# Autodesk Inventor assembly: ASY MSC Жабры
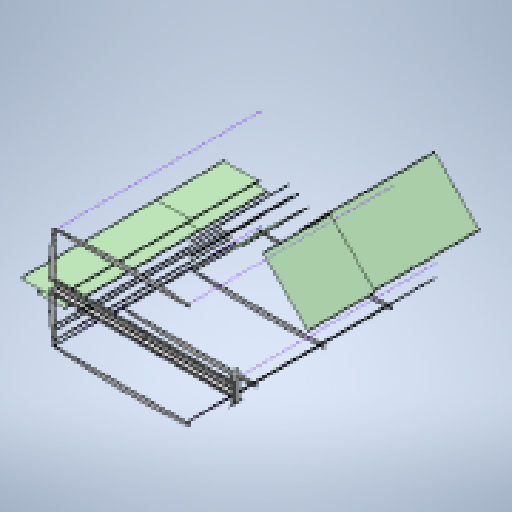
[picture p0: Inventor's stored thumbnail of the model, 512x512]
Saved by Autodesk Inventor 2025 (Build 290162010, 162A)
## iProperties
Created: 2024-08-31
Part Number: ASY MSC Жабры
Document SubType Name: Assembly
Designer: pokla
Author: pokla
## Documents named in this file (24)
- C:\Users\admin\YandexDisk-badmisterfox\домашниий пк\Inventor\Manturovo\Manturovo_Se-clar\ASY MSC Жабры.iam
- C:\Users\admin\YandexDisk-badmisterfox\домашниий пк\Inventor\Manturovo\Manturovo_Se-clar\MSC 0101 sheet gills.ipt
- C:\Users\admin\YandexDisk-badmisterfox\домашниий пк\Inventor\Manturovo\Manturovo_Se-clar\MSC 081 pillar 1.ipt
- C:\Users\admin\YandexDisk-badmisterfox\домашниий пк\Inventor\Manturovo\Manturovo_Se-clar\MSC 0102 sheet gills.ipt
- C:\Users\admin\YandexDisk-badmisterfox\домашниий пк\Inventor\Manturovo\Manturovo_Se-clar\MSC 0202 sheet gills.ipt
- C:\Users\admin\YandexDisk-badmisterfox\домашниий пк\Inventor\Manturovo\Manturovo_Se-clar\MSC 0103 sheet gills.ipt
- C:\Users\admin\YandexDisk-badmisterfox\домашниий пк\Inventor\Manturovo\Manturovo_Se-clar\MSC 0203 sheet gills.ipt
- C:\Users\admin\YandexDisk-badmisterfox\домашниий пк\Inventor\Manturovo\Manturovo_Se-clar\MSC 0104 sheet gills.ipt
- C:\Users\admin\YandexDisk-badmisterfox\домашниий пк\Inventor\Manturovo\Manturovo_Se-clar\MSC 0204 sheet gills.ipt
- C:\Users\admin\YandexDisk-badmisterfox\домашниий пк\Inventor\Manturovo\Manturovo_Se-clar\MSC 0105 sheet gills.ipt
- C:\Users\admin\YandexDisk-badmisterfox\домашниий пк\Inventor\Manturovo\Manturovo_Se-clar\MSC 0205 sheet gills.ipt
- C:\Users\admin\YandexDisk-badmisterfox\домашниий пк\Inventor\Manturovo\Manturovo_Se-clar\MSC 0106 sheet gills.ipt
- C:\Users\admin\YandexDisk-badmisterfox\домашниий пк\Inventor\Manturovo\Manturovo_Se-clar\MSC 0206 sheet gills.ipt
- C:\Users\admin\YandexDisk-badmisterfox\домашниий пк\Inventor\Manturovo\Manturovo_Se-clar\MSC 0107 sheet gills.ipt
- C:\Users\admin\YandexDisk-badmisterfox\домашниий пк\Inventor\Manturovo\Manturovo_Se-clar\MSC 0207 sheet gills.ipt
- C:\Users\admin\YandexDisk-badmisterfox\домашниий пк\Inventor\Manturovo\Manturovo_Se-clar\MSC 079 creen pillar.ipt
- C:\Users\admin\YandexDisk-badmisterfox\домашниий пк\Inventor\Manturovo\Manturovo_Se-clar\MSC DIM 085 tube belly.ipt
- C:\Users\admin\YandexDisk-badmisterfox\домашниий пк\Inventor\Manturovo\Manturovo_Se-clar\MSC 081 pillar 1_CPY.ipt
- C:\Users\admin\YandexDisk-badmisterfox\домашниий пк\Inventor\Manturovo\Manturovo_Se-clar\MSC 0211 string for sheets.ipt
- C:\Users\admin\YandexDisk-badmisterfox\домашниий пк\Inventor\Manturovo\Manturovo_Se-clar\MSC 079 top pillar.ipt
- C:\Users\admin\YandexDisk-badmisterfox\домашниий пк\Inventor\Manturovo\Manturovo_Se-clar\MSC DIM 085.1 heel.ipt
- C:\Users\admin\YandexDisk-badmisterfox\домашниий пк\Inventor\Manturovo\Manturovo_Se-clar\MSC 0201 sheet gills.ipt
- C:\Users\admin\YandexDisk-badmisterfox\домашниий пк\Inventor\Manturovo\Manturovo_Se-clar\MSC 0101 sheet gills_MIR.ipt
- C:\Users\admin\YandexDisk-badmisterfox\домашниий пк\Inventor\Manturovo\Manturovo_Se-clar\MSC 0201 sheet gills_MIR.ipt
## Components (34 placed, 23 different names)
1. MSC 0102 sheet gills:1 — Tangent:4, Tangent:5
2. MSC 0202 sheet gills:1
3. MSC 0103 sheet gills:1
4. MSC 0203 sheet gills:1
5. MSC 0104 sheet gills:1
6. MSC 0204 sheet gills:1
7. MSC 0105 sheet gills:1
8. MSC 0205 sheet gills:1
9. MSC 0106 sheet gills:1 — Rigid:21
10. MSC 0206 sheet gills:1 — Rigid:21
11. MSC 0107 sheet gills:1 — Rigid:22
12. MSC 0207 sheet gills:1 — Rigid:22
13. MSC DIM 085.1 heel:2 — Rigid:6
14. MSC DIM 085.1 heel:1 — Rigid:7
15. MSC 079 creen pillar:2 — Rigid:10, Rigid:15
16. MSC 079 top pillar:2 — Rigid:10, Rigid:24, Rigid:29
17. MSC 079 top pillar:1 — Rigid:23, Rigid:28
18. MSC 081 pillar 1_CPY:1 — Rigid:28, Rigid:29
19. MSC 079 creen pillar:1 — Rigid:12, Rigid:25
20. MSC 0211 string for sheets:2 — Rigid:12, Tangent:1, Tangent:2
21. MSC 0211 string for sheets:4 — Rigid:15
22. MSC 0211 string for sheets:1 — Rigid:13, Tangent:3
23. MSC 0211 string for sheets:3 — Rigid:16
24. MSC 0201 sheet gills_MIR:1
25. MSC 0101 sheet gills_MIR:1
26. MSC 0201 sheet gills:1 — Flush:7, Flush:8, Mate:17
27. MSC 0101 sheet gills.ipt:1 — Tangent:1, Tangent:2, Tangent:3, Flush:7, Flush:8, Mate:18
28. MSC 0211 string for sheets:143 — Rigid:23, Tangent:4, Tangent:5
29. MSC 0211 string for sheets:152 — Rigid:24
30. MSC 079 creen pillar:3 — Rigid:25, Rigid:26, Mate:17
31. MSC 079 creen pillar:4 — Rigid:26, Rigid:27
32. MSC 079 creen pillar:5 — Rigid:27, Mate:18
33. MSC DIM 085 tube belly:1 — Rigid:6, Rigid:7, Mate:11, Mate:12, Mate:13, Mate:15, Mate:16, Flush:9
34. MSC 081 pillar 1:1 — Mate:11, Mate:12, Mate:13, Rigid:13, Rigid:16
## Relationships (33: WeldJoint 17, Mate 8, Tangent 5, Flush 3)
- [Mate] (50 mm): MSC 0106 sheet gills:1 ↔ MSC 0107 sheet gills:1
- [WeldJoint]: MSC 081 pillar 1_CPY:1 ↔ MSC 081 pillar 1:1
- Rigid:6 [WeldJoint]: MSC DIM 085.1 heel:2 ↔ MSC DIM 085 tube belly:1
- Rigid:7 [WeldJoint]: MSC DIM 085.1 heel:1 ↔ MSC DIM 085 tube belly:1
- Mate:11: MSC DIM 085 tube belly:1 ↔ MSC 081 pillar 1:1
- Mate:12: MSC DIM 085 tube belly:1 ↔ MSC 081 pillar 1:1
- Mate:13: MSC DIM 085 tube belly:1 ↔ MSC 081 pillar 1:1
- Rigid:10 [WeldJoint]: MSC 079 creen pillar:2 ↔ MSC 079 top pillar:2
- Rigid:12 [WeldJoint] (-5 mm): MSC 079 creen pillar:1 ↔ MSC 0211 string for sheets:2
- Rigid:13 [WeldJoint] (-5 mm): MSC 0211 string for sheets:1 ↔ MSC 081 pillar 1:1
- Rigid:15 [WeldJoint] (-5 mm): MSC 079 creen pillar:2 ↔ MSC 0211 string for sheets:4
- Rigid:16 [WeldJoint] (-5 mm): MSC 0211 string for sheets:3 ↔ MSC 081 pillar 1:1
- Rigid:21 [WeldJoint]: MSC 0106 sheet gills:1 ↔ MSC 0206 sheet gills:1
- Rigid:22 [WeldJoint]: MSC 0107 sheet gills:1 ↔ MSC 0207 sheet gills:1
- Tangent:1: MSC 0211 string for sheets:2 ↔ MSC 0101 sheet gills.ipt:1
- Tangent:2: MSC 0211 string for sheets:2 ↔ MSC 0101 sheet gills.ipt:1
- Tangent:3: MSC 0211 string for sheets:1 ↔ MSC 0101 sheet gills.ipt:1
- Flush:7: MSC 0201 sheet gills:1 ↔ MSC 0101 sheet gills.ipt:1
- Flush:8: MSC 0201 sheet gills:1 ↔ MSC 0101 sheet gills.ipt:1
- Mate:15: MSC DIM 085 tube belly:1
- Mate:16: MSC DIM 085 tube belly:1
- Flush:9: MSC DIM 085 tube belly:1
- Rigid:23 [WeldJoint] (-5 mm): MSC 079 top pillar:1 ↔ MSC 0211 string for sheets:143
- Rigid:24 [WeldJoint] (-5 mm): MSC 079 top pillar:2 ↔ MSC 0211 string for sheets:152
- Tangent:4: MSC 0102 sheet gills:1 ↔ MSC 0211 string for sheets:143
- Tangent:5: MSC 0102 sheet gills:1 ↔ MSC 0211 string for sheets:143
- Rigid:25 [WeldJoint] (985 mm): MSC 079 creen pillar:1 ↔ MSC 079 creen pillar:3
- Rigid:26 [WeldJoint] (985 mm): MSC 079 creen pillar:3 ↔ MSC 079 creen pillar:4
- Rigid:27 [WeldJoint] (985 mm): MSC 079 creen pillar:4 ↔ MSC 079 creen pillar:5
- Rigid:28 [WeldJoint]: MSC 079 top pillar:1 ↔ MSC 081 pillar 1_CPY:1
- Rigid:29 [WeldJoint]: MSC 079 top pillar:2 ↔ MSC 081 pillar 1_CPY:1
- Mate:17: MSC 0201 sheet gills:1 ↔ MSC 079 creen pillar:3
- Mate:18: MSC 0101 sheet gills.ipt:1 ↔ MSC 079 creen pillar:5
